# Autodesk Inventor assembly: Assembly3
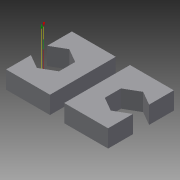
[picture p0: Inventor's stored thumbnail of the model, 180x180]
Saved by Autodesk Inventor 2015 SP1 (Build 190203100, 203)
## iProperties
Created: 2015-05-10
Part Number: Assembly3
Document SubType Name: Assembly
Designer: ubik
Author: ubik
## Documents named in this file (2)
- C:\Users\ubik\Dropbox\DueTech\cable test\Assembly3.iam
- C:\Users\ubik\Dropbox\DueTech\cable test\piulita telescop.ipt
## Components (2 placed, 1 different names)
1. piulita telescop:1 — Mate:1, Flush:1, Flush:2
2. piulita telescop:2 — Mate:1, Flush:1, Flush:2
## Relationships (3: Flush 2, Mate 1)
- Mate:1 (6.5 mm): piulita telescop:1 ↔ piulita telescop:2
- Flush:1: piulita telescop:1 ↔ piulita telescop:2
- Flush:2: piulita telescop:1 ↔ piulita telescop:2
